# Autodesk Inventor assembly: AA-Cell-x4
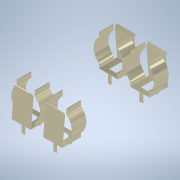
[picture p0: Inventor's stored thumbnail of the model, 180x180]
Saved by Autodesk Inventor 2022 (Build 260153000, 153)
## iProperties
Created: 2024-06-20
Part Number: AA-Cell-x4
Document SubType Name: Assembly
Designer: yamashita1
Author: yamashita1
## Documents named in this file (2)
- G:\マイドライブ\project\micro-mouse\3D-Model\AA-Cell-x2.iam
- G:\マイドライブ\project\micro-mouse\3D-Model\AA-Cell-Holder.ipt
## Components (4 placed, 1 different names)
1. AA-Cell-Holder:1 — フラッシュ:1, フラッシュ:2, メイト:1, フラッシュ:9, フラッシュ:10, フラッシュ:15
2. AA-Cell-Holder:2 — フラッシュ:1, フラッシュ:2, メイト:1
3. AA-Cell-Holder:3 — フラッシュ:9, フラッシュ:10, フラッシュ:15
4. AA-Cell-Holder:4
## Relationships (9: Flush 7, Mate 2)
- フラッシュ:1 [Flush]: AA-Cell-Holder:1 ↔ AA-Cell-Holder:2
- フラッシュ:2 [Flush]: AA-Cell-Holder:1 ↔ AA-Cell-Holder:2
- メイト:1 [Mate] (32.5 mm): AA-Cell-Holder:1 ↔ AA-Cell-Holder:2
- [Flush]: AA-Cell-Holder:3 ↔ AA-Cell-Holder:4
- [Flush]: AA-Cell-Holder:3 ↔ AA-Cell-Holder:4
- [Mate] (32.5 mm): AA-Cell-Holder:3 ↔ AA-Cell-Holder:4
- フラッシュ:9 [Flush]: AA-Cell-Holder:1 ↔ AA-Cell-Holder:3
- フラッシュ:10 [Flush]: AA-Cell-Holder:1 ↔ AA-Cell-Holder:3
- フラッシュ:15 [Flush] (15 mm): AA-Cell-Holder:1 ↔ AA-Cell-Holder:3
## Named parameters: d3_d0 = 0 mm, d4_d1 = 0 mm, d5_d2 = 32.5 mm, AA_LEN = 50.5 mm, CELL_PITCH = 15 mm
